# Autodesk Inventor assembly: Grundplatte_test
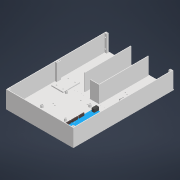
[picture p0: Inventor's stored thumbnail of the model, 180x180]
Saved by Autodesk Inventor 2021 (Build 250183000, 183)
## iProperties
Created: 2021-01-26
Part Number: Grundplatte_test
Document SubType Name: Assembly
Designer: Ctroi
Author: Ctroi
## Documents named in this file (6)
- E:\Projects\Rover\Grundplatte_test.iam
- E:\Projects\Rover\Grundplatte_hinten.ipt
- E:\Projects\Rover\Grundplatte_vorne.ipt
- E:\Projects\Rover\ArduinoMega.ipt
- E:\Projects\Rover\Relais.ipt
- E:\Projects\Rover\Kreuz_Halterung.ipt
## Components (5 placed, 5 different names)
1. Grundplatte_hinten:1 — Passend:1, Passend:2, Passend:5, Passend:6, Passend:7
2. Grundplatte_vorne:1 — Passend:1, Passend:2, Passend:3, Passend:4
3. ArduinoMega:1 — Passend:3, Passend:4
4. Relais:1
5. Kreuz_Halterung:1 — Passend:5, Passend:6, Passend:7
## Relationships (7: Mate 7)
- Passend:1 [Mate]: Grundplatte_hinten:1 ↔ Grundplatte_vorne:1
- Passend:2 [Mate]: Grundplatte_hinten:1 ↔ Grundplatte_vorne:1
- Passend:3 [Mate]: Grundplatte_vorne:1 ↔ ArduinoMega:1
- Passend:4 [Mate]: Grundplatte_vorne:1 ↔ ArduinoMega:1
- Passend:5 [Mate]: Grundplatte_hinten:1 ↔ Kreuz_Halterung:1
- Passend:6 [Mate]: Grundplatte_hinten:1 ↔ Kreuz_Halterung:1
- Passend:7 [Mate]: Grundplatte_hinten:1 ↔ Kreuz_Halterung:1
